# Autodesk Inventor assembly: Assembly1
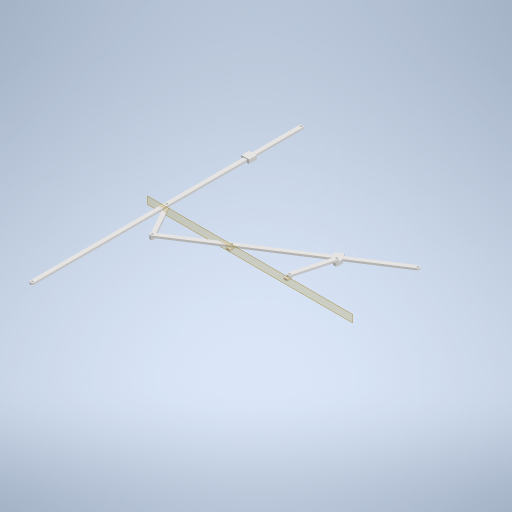
[picture p0: Inventor's stored thumbnail of the model, 512x512]
Saved by Autodesk Inventor 2024 (Build 280153000, 153)
## iProperties
Created: 2025-09-18
Part Number: Assembly1
Document SubType Name: Assembly
Designer: Hello
Author: Hello
## Documents named in this file (8)
- C:\Users\Hello\Desktop\BTMP\Assembly1.iam
- C:\Users\Hello\Desktop\BTMP\gối.ipt
- C:\Users\Hello\Desktop\BTMP\AB.ipt
- C:\Users\Hello\Desktop\BTMP\BCD.ipt
- C:\Users\Hello\Desktop\BTMP\2.ipt
- C:\Users\Hello\Desktop\BTMP\goi truot.ipt
- C:\Users\Hello\Desktop\BTMP\ED.ipt
- C:\Users\Hello\Desktop\BTMP\5.ipt
## Components (8 placed, 7 different names)
1. gối:1 — Flush:1, Mate:1, Mate:2, Mate:3, Flush:3
2. gối:2 — Flush:2, Mate:1, Mate:4, Mate:5, Mate:10
3. AB:1 — Mate:2, Mate:3, Mate:6, Mate:7, Flush:3
4. BCD:1 — Mate:4, Mate:5, Mate:8, Mate:9, Mate:11, Mate:12
5. 2:1 — Mate:6, Mate:7, Mate:8, Mate:9
6. goi truot:1 — Mate:10, Mate:15, Mate:16
7. ED:1 — Mate:11, Mate:12, Mate:13, Mate:14
8. 5:1 — Mate:13, Mate:14, Mate:15, Mate:16
## Relationships (19: Mate 16, Flush 3)
- Flush:1: gối:1
- Flush:2: gối:2
- Mate:1 (280 mm): gối:1 ↔ gối:2
- Mate:2: gối:1 ↔ AB:1
- Mate:3: gối:1 ↔ AB:1
- Mate:4: gối:2 ↔ BCD:1
- Mate:5: gối:2 ↔ BCD:1
- Mate:6: AB:1 ↔ 2:1
- Mate:7: AB:1 ↔ 2:1
- Mate:8: BCD:1 ↔ 2:1
- Mate:9: BCD:1 ↔ 2:1
- Mate:10 (320 mm): gối:2 ↔ goi truot:1
- Mate:11: BCD:1 ↔ ED:1
- Mate:12: BCD:1 ↔ ED:1
- Mate:13: ED:1 ↔ 5:1
- Mate:14: ED:1 ↔ 5:1
- Mate:15: goi truot:1 ↔ 5:1
- Mate:16: goi truot:1 ↔ 5:1
- Flush:3: gối:1 ↔ AB:1
